# Autodesk Inventor assembly: ASSEMBLY
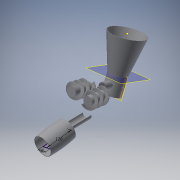
[picture p0: Inventor's stored thumbnail of the model, 180x180]
Saved by Autodesk Inventor 2019 (Build 230136000, 136)
## iProperties
Created: 2020-02-19
Part Number: ASSEMBLY
Document SubType Name: Assembly
Designer: User
Author: User
## Documents named in this file (8)
- E:\Basavraj\ASSEMBLY.iam
- C:\Users\User\Desktop\AUTODESK ENGG EXPLO\doughpush.ipt
- C:\Users\User\Desktop\AUTODESK ENGG EXPLO\outlet pipe.ipt
- C:\Users\User\Desktop\AUTODESK ENGG EXPLO\rollers.ipt
- C:\Users\User\Desktop\AUTODESK ENGG EXPLO\slide.ipt
- C:\Users\User\Desktop\AUTODESK ENGG EXPLO\sugardrum1.ipt
- C:\Users\User\Desktop\AUTODESK ENGG EXPLO\Container 1.ipt
- C:\Users\User\Desktop\AUTODESK ENGG EXPLO\Container 2.ipt
## Components (8 placed, 7 different names)
1. doughpush:1 — Mate:1, Angle:1
2. outlet pipe:1
3. rollers:1
4. rollers:2
5. slide:1
6. sugardrum1:2
7. Container 1:1
8. Container 2:1
## Relationships (2: Mate 1, Angle 1)
- Mate:1: doughpush:1
- Angle:1 (90 deg): doughpush:1
